# Autodesk Inventor assembly: Clip
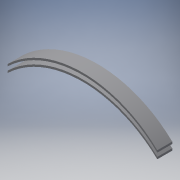
[picture p0: Inventor's stored thumbnail of the model, 180x180]
Saved by Autodesk Inventor 2016 (Build 200138000, 138)
## iProperties
Created: 2016-08-20
Part Number: Clip
Document SubType Name: Assembly
Designer: yash
Author: yash
## Documents named in this file (2)
- C:\Users\yash\Documents\GitHub\ClipFanHat\Clip.iam
- C:\Users\yash\Documents\GitHub\ClipFanHat\Clip.ipt
## Components (2 placed, 1 different names)
1. Clip:1 — Flush:1, Flush:2, Flush:3, Mate:1
2. Clip:2 — Flush:1, Flush:2, Flush:3, Mate:1
## Relationships (4: Flush 3, Mate 1)
- Flush:1: Clip:1 ↔ Clip:2
- Flush:2: Clip:1 ↔ Clip:2
- Flush:3: Clip:1 ↔ Clip:2
- Mate:1 (3.175 mm): Clip:1 ↔ Clip:2
